# Autodesk Inventor assembly: Pedestal Fixture Assembly
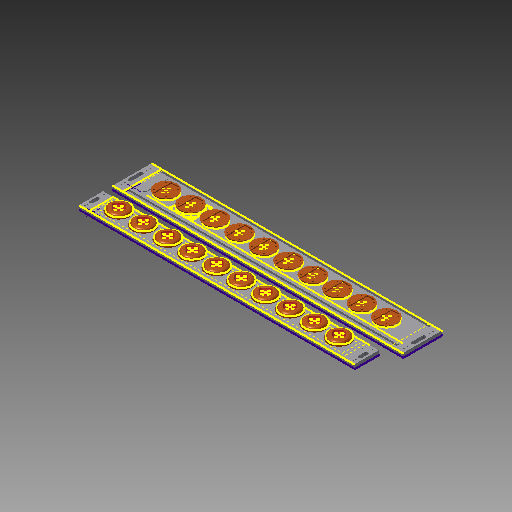
[picture p0: Inventor's stored thumbnail of the model, 512x512]
Saved by Autodesk Inventor 2018 (Build 220112000, 112)
## iProperties
Created: 2017-07-11
Part Number: Pedestal Fixture Assembly
Document SubType Name: Assembly
Designer: Samuel Clay
Author: Samuel Clay
## Documents named in this file (3)
- Z:\enclosure\inventor\Pedestal Fixture Assembly.iam
- Z:\enclosure\inventor\Pedestal Fixture Base.ipt
- Z:\enclosure\inventor\Pedestal.ipt
## Components (21 placed, 2 different names)
1. Pedestal Fixture Base:1 — Mate:1, Mate:2, Mate:3, Mate:9, Mate:10, Mate:11
2. Pedestal:2 — Mate:1, Mate:2, Mate:3
3. Pedestal:3
4. Pedestal:4
5. Pedestal:5
6. Pedestal:15
7. Pedestal:16
8. Pedestal:17
9. Pedestal:18
10. Pedestal:19
11. Pedestal:20
12. Pedestal:1 — Mate:9, Mate:10, Mate:11
13. Pedestal:6
14. Pedestal:7
15. Pedestal:8
16. Pedestal:9
17. Pedestal:10
18. Pedestal:11
19. Pedestal:12
20. Pedestal:13
21. Pedestal:14
## Component patterns: (10 elements, first: Pedestal:2), (10 elements, first: Pedestal:1)
## Relationships (6: Mate 6)
- Mate:1 (0.635 mm): Pedestal Fixture Base:1 ↔ Pedestal:2
- Mate:2 (3.81 mm): Pedestal Fixture Base:1 ↔ Pedestal:2
- Mate:3 (2.54 mm): Pedestal Fixture Base:1 ↔ Pedestal:2
- Mate:9 (15.24 mm): Pedestal Fixture Base:1 ↔ Pedestal:1
- Mate:10 (-38.1 mm): Pedestal Fixture Base:1 ↔ Pedestal:1
- Mate:11 (-6.35 mm): Pedestal Fixture Base:1 ↔ Pedestal:1
